# Autodesk Inventor assembly: rubber wheels and motor
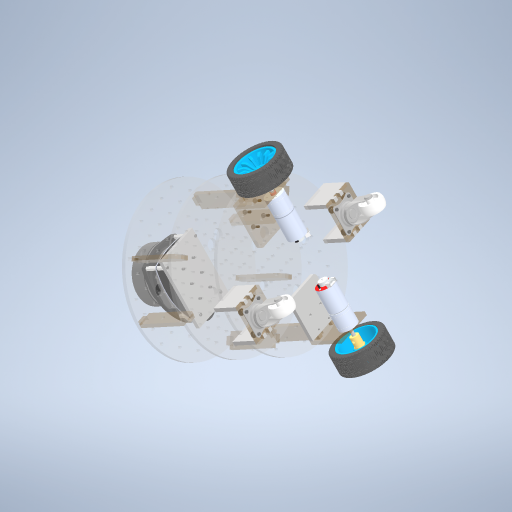
[picture p0: Inventor's stored thumbnail of the model, 512x512]
Saved by Autodesk Inventor 2023.2 (Build 272271000, 271)
## iProperties
Created: 2024-08-13
Part Number: rubber wheels and motor
Document SubType Name: Assembly
Designer: PC
Author: PC
## Documents named in this file (15)
- C:\Users\PC\Desktop\rubber wheels and motor.iam
- C:\Users\PC\Desktop\65mm蓝色轮胎总装-实际外径68mm.iam
- C:\Users\PC\Desktop\Motor.ipt
- C:\Users\PC\Desktop\motor wheel connector.ipt
- C:\Users\PC\Desktop\Kinghts mobile platform\Knights Mobile platform design.iam
- C:\Users\PC\Documents\Inventor\Content Center Files\R2023\en-US\ISO 1580\ISO 1580 - M3 x 8_.ipt
- C:\Users\PC\Desktop\motor wheel assembly2.iam
- C:\Users\PC\Desktop\Caster-swivel-40mm_assembly\Caster-swivel-40mm_assembly.iam
- C:\Users\PC\Desktop\caster wheel mounter.ipt
- C:\Users\PC\Documents\Inventor\Content Center Files\R2023\en-US\ISO 1580\ISO 1580 - M4 x 8_.ipt
- C:\Users\PC\Desktop\RP-lidar-A1\RP-lidar-A1.iam
- C:\Users\PC\Documents\Inventor\Content Center Files\R2023\en-US\ISO 1580\ISO 1580 - M2 x 12_.ipt
- C:\Users\PC\Desktop\Kinghts mobile platform\custom standoffs.ipt
- C:\Users\PC\Desktop\Kinghts mobile platform\motorchassisholder2Ass.iam
- C:\Users\PC\Desktop\Kinghts mobile platform\casterholderA.ipt
## Components (39 placed, 14 different names)
1. Knights Mobile platform design:1 [sub-assembly] — Insert:7, Insert:8, Insert:9, Insert:10, Insert:15, Insert:16, Insert:17, Insert:18, Flush:1, Flush:2, Mate:1, Flush:3, Flush:4, Mate:2, Insert:40, Insert:41, Insert:42, Insert:43, Flush:5, Flush:6, Mate:3, Flush:7, Flush:8, Mate:4, Flush:9, Mate:5, Mate:6, Flush:10, Flush:11, Mate:7, Insert:46, Insert:47, Insert:49, Insert:50, Flush:12, Mate:8, Flush:13, Flush:14, Mate:9, Flush:15, Flush:16, Flush:17, Mate:10, Flush:18, Mate:11
2. 65mm蓝色轮胎总装-实际外径68mm:2 [sub-assembly]
3. Motor:2 — Insert:48
4. motor wheel connector:2
5. ISO 1580 M3 x 8:1 — Insert:15, Insert:21
6. ISO 1580 M3 x 8:2 — Insert:16, Insert:20
7. ISO 1580 M3 x 8:3 — Insert:10
8. ISO 1580 M3 x 8:4 — Insert:7
9. ISO 1580 M3 x 8:5 — Insert:8
10. ISO 1580 M3 x 8:6 — Insert:9
11. ISO 1580 M3 x 8:7 — Insert:17, Insert:22
12. ISO 1580 M3 x 8:8 — Insert:18, Insert:19
13. motor wheel assembly2:1 [sub-assembly] — Insert:19, Insert:20, Insert:21, Insert:22, Insert:46, Insert:47
14. Caster-swivel-40mm_assembly:1 [sub-assembly] — Insert:27, Insert:28, Insert:38, Insert:39
15. Caster-swivel-40mm_assembly:2 [sub-assembly] — Insert:36, Insert:37
16. caster wheel mounter:1 — Flush:1, Flush:2, Mate:1, Insert:24, Insert:25, Insert:29, Insert:30
17. caster wheel mounter:2 — Flush:3, Flush:4, Mate:2, Insert:32, Insert:33, Insert:34, Insert:35
18. ISO 1580 M4 x 8:1 — Insert:33
19. ISO 1580 M4 x 8:2 — Insert:32, Insert:36
20. ISO 1580 M4 x 8:3 — Insert:25, Insert:28, Insert:38
21. ISO 1580 M4 x 8:4 — Insert:30
22. ISO 1580 M4 x 8:5 — Insert:24, Insert:27
23. ISO 1580 M4 x 8:6 — Insert:34, Insert:37
24. ISO 1580 M4 x 8:7 — Insert:29, Insert:39
25. ISO 1580 M4 x 8:8 — Insert:35
26. RP-lidar-A1:1 [sub-assembly] — Insert:44, Insert:45
27. ISO 1580 M2 x 12:1 — Insert:43
28. ISO 1580 M2 x 12:2 — Insert:41, Insert:44
29. ISO 1580 M2 x 12:3 — Insert:40, Insert:45
30. ISO 1580 M2 x 12:4 — Insert:42
31. custom standoffs:1 — Flush:7, Flush:8, Mate:4
32. custom standoffs:2 — Flush:5, Flush:6, Mate:3
33. custom standoffs:3 — Flush:9, Mate:5, Mate:6
34. custom standoffs:4 — Flush:10, Flush:11, Mate:7
35. motorchassisholder2Ass:1 [sub-assembly] — Insert:48, Insert:49, Insert:50
36. casterholderA:1 — Flush:12, Mate:8, Flush:13
37. casterholderA:2 — Flush:14, Mate:9, Flush:15
38. casterholderA:3 — Flush:18, Mate:11
39. casterholderA:4 — Flush:16, Flush:17, Mate:10
## Relationships (68: Insert 39, Flush 18, Mate 11)
- [Insert] (-9 mm): Motor:2 ↔ motor wheel connector:2
- [Insert] (-12 mm): 65mm蓝色轮胎总装-实际外径68mm:2 ↔ motor wheel connector:2
- Insert:7 (-7.8 mm): Knights Mobile platform design:1 ↔ ISO 1580 M3 x 8:4
- Insert:8 (-7.8 mm): Knights Mobile platform design:1 ↔ ISO 1580 M3 x 8:5
- Insert:9 (-7.8 mm): Knights Mobile platform design:1 ↔ ISO 1580 M3 x 8:6
- Insert:10 (-7.8 mm): Knights Mobile platform design:1 ↔ ISO 1580 M3 x 8:3
- Insert:15 (-7.8 mm): Knights Mobile platform design:1 ↔ ISO 1580 M3 x 8:1
- Insert:16 (-7.8 mm): Knights Mobile platform design:1 ↔ ISO 1580 M3 x 8:2
- Insert:17 (-7.8 mm): Knights Mobile platform design:1 ↔ ISO 1580 M3 x 8:7
- Insert:18 (-7.8 mm): Knights Mobile platform design:1 ↔ ISO 1580 M3 x 8:8
- Insert:19 (-2.9 mm): ISO 1580 M3 x 8:8 ↔ motor wheel assembly2:1
- Insert:20 (-2.9 mm): ISO 1580 M3 x 8:2 ↔ motor wheel assembly2:1
- Insert:21 (-2.9 mm): ISO 1580 M3 x 8:1 ↔ motor wheel assembly2:1
- Insert:22 (-2.9 mm): ISO 1580 M3 x 8:7 ↔ motor wheel assembly2:1
- Flush:1 (-50.34 mm): Knights Mobile platform design:1 ↔ caster wheel mounter:1
- Flush:2: Knights Mobile platform design:1 ↔ caster wheel mounter:1
- Mate:1: Knights Mobile platform design:1 ↔ caster wheel mounter:1
- Insert:24 (-7.8 mm): caster wheel mounter:1 ↔ ISO 1580 M4 x 8:5
- Insert:25 (-7.8 mm): caster wheel mounter:1 ↔ ISO 1580 M4 x 8:3
- Insert:27 (-2.9 mm): Caster-swivel-40mm_assembly:1 ↔ ISO 1580 M4 x 8:5
- Insert:28 (-2.9 mm): Caster-swivel-40mm_assembly:1 ↔ ISO 1580 M4 x 8:3
- Insert:29 (-7.8 mm): caster wheel mounter:1 ↔ ISO 1580 M4 x 8:7
- Insert:30 (-7.8 mm): caster wheel mounter:1 ↔ ISO 1580 M4 x 8:4
- Flush:3: Knights Mobile platform design:1 ↔ caster wheel mounter:2
- Flush:4 (-50.34 mm): Knights Mobile platform design:1 ↔ caster wheel mounter:2
- Mate:2: Knights Mobile platform design:1 ↔ caster wheel mounter:2
- Insert:32 (-7.8 mm): caster wheel mounter:2 ↔ ISO 1580 M4 x 8:2
- Insert:33 (-7.8 mm): caster wheel mounter:2 ↔ ISO 1580 M4 x 8:1
- Insert:34 (-7.8 mm): caster wheel mounter:2 ↔ ISO 1580 M4 x 8:6
- Insert:35 (-7.8 mm): caster wheel mounter:2 ↔ ISO 1580 M4 x 8:8
- Insert:36 (-2.9 mm): Caster-swivel-40mm_assembly:2 ↔ ISO 1580 M4 x 8:2
- Insert:37 (-2.9 mm): Caster-swivel-40mm_assembly:2 ↔ ISO 1580 M4 x 8:6
- Insert:38 (-2.9 mm): Caster-swivel-40mm_assembly:1 ↔ ISO 1580 M4 x 8:3
- Insert:39 (-2.9 mm): Caster-swivel-40mm_assembly:1 ↔ ISO 1580 M4 x 8:7
- Insert:40 (-12 mm): Knights Mobile platform design:1 ↔ ISO 1580 M2 x 12:3
- Insert:41 (-12 mm): Knights Mobile platform design:1 ↔ ISO 1580 M2 x 12:2
- Insert:42 (-12 mm): Knights Mobile platform design:1 ↔ ISO 1580 M2 x 12:4
- Insert:43 (-12 mm): Knights Mobile platform design:1 ↔ ISO 1580 M2 x 12:1
- Insert:44 (-6.9 mm): RP-lidar-A1:1 ↔ ISO 1580 M2 x 12:2
- Insert:45 (-6.9 mm): RP-lidar-A1:1 ↔ ISO 1580 M2 x 12:3
- Flush:5 (-64.2 mm): Knights Mobile platform design:1 ↔ custom standoffs:2
- Flush:6 (-5 mm): Knights Mobile platform design:1 ↔ custom standoffs:2
- Mate:3: Knights Mobile platform design:1 ↔ custom standoffs:2
- Flush:7 (-64.2 mm): Knights Mobile platform design:1 ↔ custom standoffs:1
- Flush:8 (-5 mm): Knights Mobile platform design:1 ↔ custom standoffs:1
- Mate:4: Knights Mobile platform design:1 ↔ custom standoffs:1
- Flush:9 (-64.2 mm): Knights Mobile platform design:1 ↔ custom standoffs:3
- Mate:5: Knights Mobile platform design:1 ↔ custom standoffs:3
- Mate:6: Knights Mobile platform design:1 ↔ custom standoffs:3
- Flush:10 (-64.2 mm): Knights Mobile platform design:1 ↔ custom standoffs:4
- Flush:11 (-5 mm): Knights Mobile platform design:1 ↔ custom standoffs:4
- Mate:7: Knights Mobile platform design:1 ↔ custom standoffs:4
- Insert:46: Knights Mobile platform design:1 ↔ motor wheel assembly2:1
- Insert:47: Knights Mobile platform design:1 ↔ motor wheel assembly2:1
- Insert:48 (-2.35 mm): Motor:2 ↔ motorchassisholder2Ass:1
- Insert:49: Knights Mobile platform design:1 ↔ motorchassisholder2Ass:1
- Insert:50: Knights Mobile platform design:1 ↔ motorchassisholder2Ass:1
- Flush:12 (-5.2 mm): Knights Mobile platform design:1 ↔ casterholderA:1
- Mate:8: Knights Mobile platform design:1 ↔ casterholderA:1
- Flush:13: Knights Mobile platform design:1 ↔ casterholderA:1
- Flush:14: Knights Mobile platform design:1 ↔ casterholderA:2
- Mate:9: Knights Mobile platform design:1 ↔ casterholderA:2
- Flush:15 (-5.2 mm): Knights Mobile platform design:1 ↔ casterholderA:2
- Flush:16 (-5.2 mm): Knights Mobile platform design:1 ↔ casterholderA:4
- Flush:17: Knights Mobile platform design:1 ↔ casterholderA:4
- Mate:10: Knights Mobile platform design:1 ↔ casterholderA:4
- Flush:18: Knights Mobile platform design:1 ↔ casterholderA:3
- Mate:11: Knights Mobile platform design:1 ↔ casterholderA:3
## Named parameters: d4_d0 = -9 mm, d6_d1 = -12 mm
